# Autodesk Inventor assembly: ujj_alapmodell
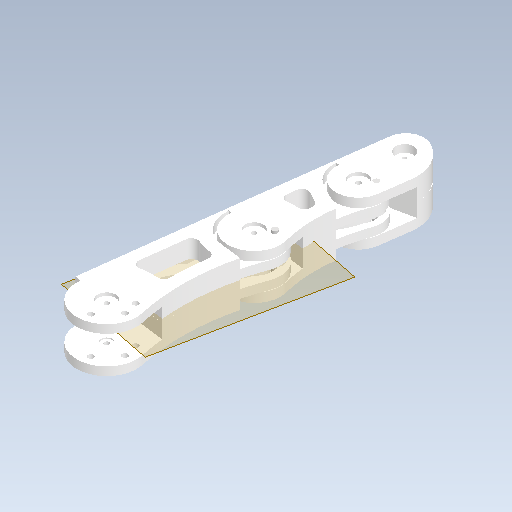
[picture p0: Inventor's stored thumbnail of the model, 512x512]
Saved by Autodesk Inventor 2020.3 (Build 243373000, 373)
## iProperties
Created: 2019-08-09
Part Number: ujj_alapmodell
Document SubType Name: Assembly
Designer: Horváth Patrik
Author: Horváth Patrik
## Documents named in this file (11)
- E:\Dokumentumok\Simonyi\INDACT\Robotarm - kézfej fileok\kéz12.0\ujj_alapmodell.iam
- E:\Dokumentumok\Simonyi\INDACT\Robotarm - kézfej fileok\kéz12.0\Solid1.ipt
- E:\Dokumentumok\Simonyi\INDACT\Robotarm - kézfej fileok\kéz12.0\Solid2.ipt
- E:\Dokumentumok\Simonyi\INDACT\Robotarm - kézfej fileok\kéz12.0\Solid3.ipt
- E:\Dokumentumok\Simonyi\INDACT\Robotarm - kézfej fileok\kéz12.0\Solid5.ipt
- E:\Dokumentumok\Simonyi\INDACT\Robotarm - kézfej fileok\kéz12.0\Solid6.ipt
- E:\Dokumentumok\Simonyi\INDACT\Robotarm - kézfej fileok\kéz12.0\Solid11.ipt
- E:\Dokumentumok\Simonyi\INDACT\Robotarm - kézfej fileok\kéz12.0\Solid10.ipt
- E:\Dokumentumok\Simonyi\INDACT\Robotarm - kézfej fileok\kéz12.0\Solid1_MIR1.ipt
- E:\Dokumentumok\Simonyi\INDACT\Robotarm - kézfej fileok\kéz12.0\Solid2_MIR2.ipt
- E:\Dokumentumok\Simonyi\INDACT\Robotarm - kézfej fileok\kéz12.0\Solid3_MIR2.ipt
## Components (12 placed, 10 different names)
1. Solid1:1 — Mate:8, Mate:9, Angle:1, Mate:29, Mate:34
2. Solid2:1 — Mate:8, Mate:9, Mate:16, Mate:17, Angle:1, Mate:32
3. Solid3:1 — Mate:16, Mate:17, Mate:35, Flush:9
4. Solid5:1 — Mate:29, Mate:32, Mate:33, Flush:7, Flush:8
5. Solid6:1 — Flush:8, Mate:34, Mate:35, Mate:36, Mate:37, Flush:10
6. Solid11:1
7. Solid10:1 — Mate:33, Flush:7
8. Solid11:2 — Mate:36, Flush:9
9. Solid10:2 — Mate:37, Flush:10
10. Solid1_MIR1:1
11. Solid2_MIR2:1 — Mate:38
12. Solid3_MIR2:1 — Mate:38
## Relationships (17: Mate 12, Flush 4, Angle 1)
- Mate:8: Solid1:1 ↔ Solid2:1
- Mate:9: Solid1:1 ↔ Solid2:1
- Mate:16: Solid2:1 ↔ Solid3:1
- Mate:17: Solid2:1 ↔ Solid3:1
- Angle:1 (2 deg): Solid1:1 ↔ Solid2:1
- Mate:29 (0.5 mm): Solid1:1 ↔ Solid5:1
- Mate:32: Solid2:1 ↔ Solid5:1
- Mate:33: Solid5:1 ↔ Solid10:1
- Flush:7 (-2.5 mm): Solid5:1 ↔ Solid10:1
- Flush:8: Solid5:1 ↔ Solid6:1
- Mate:34: Solid1:1 ↔ Solid6:1
- Mate:35: Solid3:1 ↔ Solid6:1
- Mate:36: Solid6:1 ↔ Solid11:2
- Flush:9: Solid3:1 ↔ Solid11:2
- Mate:37: Solid6:1 ↔ Solid10:2
- Flush:10 (-2.5 mm): Solid6:1 ↔ Solid10:2
- Mate:38: Solid2_MIR2:1 ↔ Solid3_MIR2:1
